# Autodesk Inventor assembly: rib 9 test
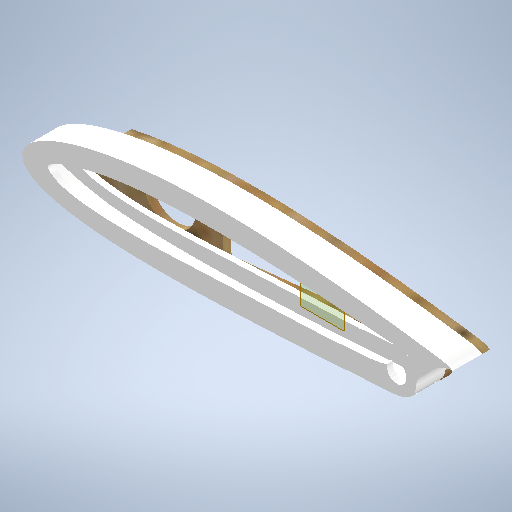
[picture p0: Inventor's stored thumbnail of the model, 512x512]
Saved by Autodesk Inventor 2025.1 (Build 291241000, 241)
## iProperties
Created: 2025-01-31
Part Number: rib 9 test
Document SubType Name: Assembly
Designer: johan
Author: johan
## Documents named in this file (3)
- C:\Users\johan\OneDrive - University of Bristol\CAD docs\2) Wing\2) Ribs\rib 9 test.iam
- C:\Users\johan\OneDrive - University of Bristol\CAD docs\2) Wing\2) Ribs\parts\Flap ribs\3P.03.09.01.JS.rib 9 ply.ipt
- C:\Users\johan\OneDrive - University of Bristol\CAD docs\2) Wing\2) Ribs\parts\Flap ribs\3P.03.09.02.JS.rib 9 foam.ipt
## Components (2 placed, 2 different names)
1. 3P.03.09.01.JS.rib 9 ply:1 — Mate:1
2. 3P.03.09.02.JS.rib 9 foam:1 — Mate:1
## Relationships (1: Mate 1)
- Mate:1: 3P.03.09.01.JS.rib 9 ply:1 ↔ 3P.03.09.02.JS.rib 9 foam:1
